# Autodesk Inventor assembly: IR_Platine
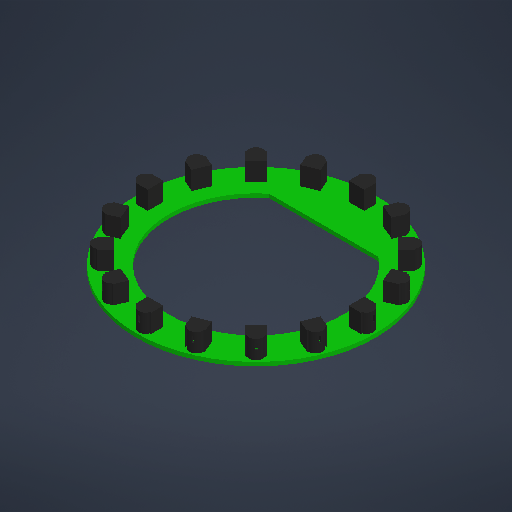
[picture p0: Inventor's stored thumbnail of the model, 512x512]
Saved by Autodesk Inventor 2025.3 (Build 293356000, 356)
## iProperties
Created: 2025-05-27
Part Number: IR_Platine
Document SubType Name: Assembly
Designer: theod
Author: theod
## Documents named in this file (3)
- C:\Users\theod\Desktop\Robotik Inventor Alles schön\IR_Platine.iam
- C:\Users\theod\Nextcloud\Inventor\2vs2 LWL Int. 2025\IR V1.ipt
- C:\Users\theod\Desktop\Robotik Inventor Alles schön\IR_Kappen.ipt
## Components (17 placed, 2 different names)
1. IR V1:1 — Passend:1, Fluchtend:1, Fluchtend:2, Passend:2
2. IR_Kappen:1 — Passend:2, Passend:3, Passend:4
3. IR_Kappen:2
4. IR_Kappen:3
5. IR_Kappen:4
6. IR_Kappen:5
7. IR_Kappen:6
8. IR_Kappen:7
9. IR_Kappen:8
10. IR_Kappen:9
11. IR_Kappen:10
12. IR_Kappen:11
13. IR_Kappen:12
14. IR_Kappen:13
15. IR_Kappen:14
16. IR_Kappen:15
17. IR_Kappen:16
## Component patterns: (16 elements, first: IR_Kappen:1)
## Relationships (6: Mate 4, Flush 2)
- Passend:1 [Mate]: IR V1:1
- Fluchtend:1 [Flush]: IR V1:1
- Fluchtend:2 [Flush]: IR V1:1
- Passend:2 [Mate]: IR V1:1 ↔ IR_Kappen:1
- Passend:3 [Mate]: IR_Kappen:1
- Passend:4 [Mate] (-55 mm): IR_Kappen:1
